# Autodesk Inventor assembly: chwytak doł
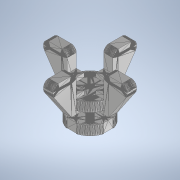
[picture p0: Inventor's stored thumbnail of the model, 180x180]
Saved by Autodesk Inventor 2022.3 (Build 263350000, 350)
## iProperties
Created: 2023-06-03
Part Number: chwytak doł
Document SubType Name: Assembly
Designer: komputer
Author: komputer
## Documents named in this file (5)
- C:\Users\komputer\Documents\Inventor\chwytak\chwytak doł.iam
- C:\Users\komputer\AppData\Local\Temp\Rar$DIa7596.38510\GripperBaseCircularLower.ipt
- C:\Users\komputer\AppData\Local\Temp\Rar$DIa7596.38510\GripperBaseCircularUpper.ipt
- C:\Users\komputer\AppData\Local\Temp\Rar$DIa7596.38510\CircularStandOff.ipt
- C:\Users\komputer\AppData\Local\Temp\Rar$DIa7596.38510\ClawShoulder.ipt
## Components (10 placed, 4 different names)
1. GripperBaseCircularLower:1 — Mate:1, Mate:2, Mate:3, Mate:4, Mate:5, Mate:6, Mate:7, Mate:8, Mate:9
2. GripperBaseCircularUpper:1 — Mate:10, Mate:11, Mate:12, Mate:13, Mate:14, Mate:15, Mate:16, Mate:17, Mate:18, Mate:19, Mate:20, Mate:21, Mate:22, Mate:23, Mate:24
3. CircularStandOff:1 — Mate:1, Mate:5, Mate:11
4. CircularStandOff:2 — Mate:2, Mate:6
5. CircularStandOff:3 — Mate:3, Mate:8, Mate:9, Mate:12
6. CircularStandOff:4 — Mate:4, Mate:7, Mate:10
7. ClawShoulder:1 — Mate:13, Mate:14, Mate:15
8. ClawShoulder:2 — Mate:16, Mate:17, Mate:18
9. ClawShoulder:3 — Mate:19, Mate:22, Mate:23
10. ClawShoulder:4 — Mate:20, Mate:21, Mate:24
## Relationships (24: Mate 24)
- Mate:1: GripperBaseCircularLower:1 ↔ CircularStandOff:1
- Mate:2: GripperBaseCircularLower:1 ↔ CircularStandOff:2
- Mate:3: GripperBaseCircularLower:1 ↔ CircularStandOff:3
- Mate:4: GripperBaseCircularLower:1 ↔ CircularStandOff:4
- Mate:5: GripperBaseCircularLower:1 ↔ CircularStandOff:1
- Mate:6: GripperBaseCircularLower:1 ↔ CircularStandOff:2
- Mate:7: GripperBaseCircularLower:1 ↔ CircularStandOff:4
- Mate:8: GripperBaseCircularLower:1 ↔ CircularStandOff:3
- Mate:9: GripperBaseCircularLower:1 ↔ CircularStandOff:3
- Mate:10: GripperBaseCircularUpper:1 ↔ CircularStandOff:4
- Mate:11: GripperBaseCircularUpper:1 ↔ CircularStandOff:1
- Mate:12: GripperBaseCircularUpper:1 ↔ CircularStandOff:3
- Mate:13: GripperBaseCircularUpper:1 ↔ ClawShoulder:1
- Mate:14: GripperBaseCircularUpper:1 ↔ ClawShoulder:1
- Mate:15: GripperBaseCircularUpper:1 ↔ ClawShoulder:1
- Mate:16: GripperBaseCircularUpper:1 ↔ ClawShoulder:2
- Mate:17: GripperBaseCircularUpper:1 ↔ ClawShoulder:2
- Mate:18: GripperBaseCircularUpper:1 ↔ ClawShoulder:2
- Mate:19: GripperBaseCircularUpper:1 ↔ ClawShoulder:3
- Mate:20: GripperBaseCircularUpper:1 ↔ ClawShoulder:4
- Mate:21: GripperBaseCircularUpper:1 ↔ ClawShoulder:4
- Mate:22: GripperBaseCircularUpper:1 ↔ ClawShoulder:3
- Mate:23: GripperBaseCircularUpper:1 ↔ ClawShoulder:3
- Mate:24: GripperBaseCircularUpper:1 ↔ ClawShoulder:4
